# Autodesk Inventor assembly: AliCe_TFT
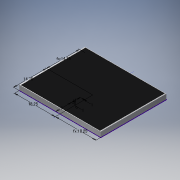
[picture p0: Inventor's stored thumbnail of the model, 180x180]
Saved by Autodesk Inventor 2016 (Build 200138000, 138)
## iProperties
Created: 2017-04-02
Part Number: AliCe_TFT
Material: 一般
Document SubType Name: Assembly
Designer: kota
Author: kota
## Documents named in this file (3)
- C:\Users\KOTA-NPC2\Dropbox\AliCe関連\MicroMouse2016\AliCe_TFT.iam
- C:\Users\KOTA-NPC2\Dropbox\AliCe関連\MicroMouse2016\TFT.ipt
- C:\Users\KOTA-NPC2\Dropbox\AliCe関連\MicroMouse2016\TFT_case.ipt
## Components (2 placed, 2 different names)
1. TFT:1 — リジッド:1
2. TFT_case:1 — リジッド:1
## Relationships (1: WeldJoint 1)
- リジッド:1 [WeldJoint]: TFT:1 ↔ TFT_case:1
